# Autodesk Inventor assembly: 3_left_leg_true_final
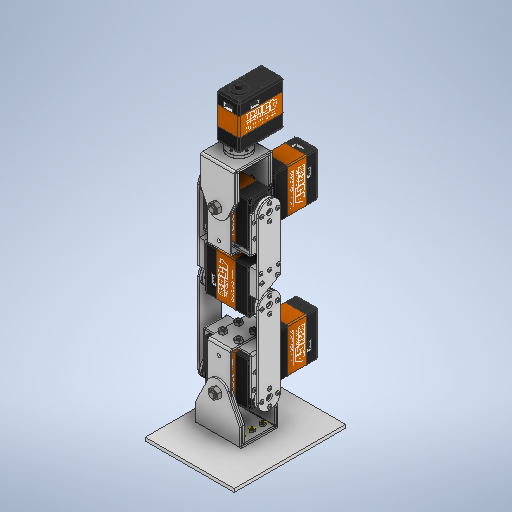
[picture p0: Inventor's stored thumbnail of the model, 512x512]
Saved by Autodesk Inventor 2026.1 (Build 301233000, 233)
## iProperties
Created: 2025-08-03
Part Number: 3_left_leg_true_final
Document SubType Name: Assembly
Designer: User
Author: User
## Documents named in this file (29)
- C:\Users\User\Documents\The Maverick's Files\College 3-3\로보인 프로젝트\RHp_Humanoid_ver1\Assembly\3_left_leg_true_final.iam
- C:\Users\User\Documents\The Maverick's Files\College 3-3\로보인 프로젝트\RHp_Humanoid_ver1\Part\HTD-45H, Horn\HTD-45H\HTD-45H.iam
- C:\Users\User\Documents\The Maverick's Files\College 3-3\로보인 프로젝트\RHp_Humanoid_ver1\Part\Frame\Leg\Left Leg\axis_1_top_frame.ipt
- C:\Users\User\Documents\The Maverick's Files\College 3-3\로보인 프로젝트\RHp_Humanoid_ver1\Part\Frame\Leg\Left Leg\axis_3_bottom_frame.ipt
- C:\Users\User\Documents\The Maverick's Files\College 3-3\로보인 프로젝트\RHp_Humanoid_ver1\Part\Frame\Leg\Left Leg\axis_2_bottom_frame.ipt
- C:\Users\User\Documents\The Maverick's Files\College 3-3\로보인 프로젝트\RHp_Humanoid_ver1\Part\Frame\Leg\Left Leg\axis_1_supplement_frame.ipt
- C:\Users\User\Documents\The Maverick's Files\College 3-3\로보인 프로젝트\RHp_Humanoid_ver1\Part\Frame\Leg\Left Leg\axis_2_4_connector_frame_powered.ipt
- C:\Users\User\Documents\The Maverick's Files\College 3-3\로보인 프로젝트\RHp_Humanoid_ver1\Part\Frame\Leg\Left Leg\axis_2_4_connector_frame_non_powered.ipt
- C:\Users\User\Documents\The Maverick's Files\College 3-3\로보인 프로젝트\RHp_Humanoid_ver1\Part\Frame\Leg\3D_printed_part_powered.ipt
- C:\Users\User\Documents\The Maverick's Files\College 3-3\로보인 프로젝트\RHp_Humanoid_ver1\Part\Frame\Leg\3D_printed_part_non_powered.ipt
- C:\Users\User\Documents\The Maverick's Files\College 3-3\로보인 프로젝트\RHp_Humanoid_ver1\Part\Frame\Leg\Left Leg\axis_4_5_connector_frame_powered.ipt
- C:\Users\User\Documents\The Maverick's Files\College 3-3\로보인 프로젝트\RHp_Humanoid_ver1\Part\Frame\Leg\Left Leg\axis_4_5_connector_frame_non_powered.ipt
- C:\Users\User\Documents\The Maverick's Files\College 3-3\로보인 프로젝트\RHp_Humanoid_ver1\Part\Frame\Leg\Left Leg\axis_5_top_frame.ipt
- C:\Users\User\Documents\The Maverick's Files\College 3-3\로보인 프로젝트\RHp_Humanoid_ver1\Part\Frame\Leg\Left Leg\axis_6_top_frame.ipt
- C:\Users\User\Documents\The Maverick's Files\College 3-3\로보인 프로젝트\RHp_Humanoid_ver1\Part\Frame\Leg\Left Leg\axis_6_bottom_frame(top).ipt
- C:\Users\User\Documents\The Maverick's Files\College 3-3\로보인 프로젝트\RHp_Humanoid_ver1\Part\Frame\Leg\Left Leg\axis_6_bottom_frame(bottom).ipt
- C:\Users\User\Documents\The Maverick's Files\College 3-3\로보인 프로젝트\RHp_Humanoid_ver1\Part\Frame\Leg\Left Leg\axis_6_supplement_frame.ipt
- C:\Users\User\Documents\The Maverick's Files\College 3-3\로보인 프로젝트\RHp_Humanoid_ver1\Part\Bolt, Bearing, Nut, Washer\볼트, 너트\볼트, 너트\M5x10 Bolt.ipt
- C:\Users\User\Documents\The Maverick's Files\College 3-3\로보인 프로젝트\RHp_Humanoid_ver1\Part\Bolt, Bearing, Nut, Washer\볼트, 너트\볼트, 너트\M5 Nylon Nut.ipt
- C:\Users\User\Documents\The Maverick's Files\College 3-3\로보인 프로젝트\RHp_Humanoid_ver1\Part\Bolt, Bearing, Nut, Washer\볼트, 너트\볼트, 너트\M3x6 Bolt.ipt
- C:\Users\User\Documents\The Maverick's Files\College 3-3\로보인 프로젝트\RHp_Humanoid_ver1\Part\Bolt, Bearing, Nut, Washer\볼트, 너트\볼트, 너트\M3 Nut.ipt
- C:\Users\User\Documents\The Maverick's Files\College 3-3\로보인 프로젝트\RHp_Humanoid_ver1\Part\Bolt, Bearing, Nut, Washer\볼트, 너트\볼트, 너트\M2x6 Bolt.ipt
- C:\Users\User\Documents\The Maverick's Files\College 3-3\로보인 프로젝트\RHp_Humanoid_ver1\Part\Bolt, Bearing, Nut, Washer\볼트, 너트\볼트, 너트\M2x4 Bolt.ipt
- C:\Users\User\Documents\The Maverick's Files\College 3-3\로보인 프로젝트\RHp_Humanoid_ver1\Part\Bolt, Bearing, Nut, Washer\볼트, 너트\볼트, 너트\M2x12 Bolt.ipt
- C:\Users\User\Documents\The Maverick's Files\College 3-3\로보인 프로젝트\RHp_Humanoid_ver1\Part\Bolt, Bearing, Nut, Washer\볼트, 너트\볼트, 너트\M2x8접시.ipt
- C:\Users\User\Documents\The Maverick's Files\College 3-3\로보인 프로젝트\RHp_Humanoid_ver1\Part\Bolt, Bearing, Nut, Washer\볼트, 너트\볼트, 너트\M2x45 Bolt.ipt
- C:\Users\User\Documents\The Maverick's Files\College 3-3\로보인 프로젝트\RHp_Humanoid_ver1\Part\HTD-45H, Horn (Silver)\HTD-45H, Horn (Silver)\Horn\Top Horn.ipt
- C:\Users\User\Documents\The Maverick's Files\College 3-3\로보인 프로젝트\RHp_Humanoid_ver1\Part\HTD-45H, Horn (Silver)\HTD-45H, Horn (Silver)\Horn\Bottom Horn.ipt
- C:\Users\User\Documents\The Maverick's Files\College 3-3\로보인 프로젝트\RHp_Humanoid_ver1\Part\Bolt, Bearing, Nut, Washer\M2 Nut.ipt
## Components (134 placed, 28 different names)
1. HTD-45H:1 [sub-assembly] — Rotational:1
2. Top Horn:1 — Rotational:1, Rigid:127
3. axis_1_top_frame:1 — Rigid:5, Rigid:29, Rigid:127, Rigid:131
4. axis_1_supplement_frame:1 — Rigid:5, Rigid:28, Rigid:83, Rigid:80, Rigid:81, Rigid:82, Rigid:84, Rigid:85, Rigid:86, Rigid:87
5. HTD-45H:3 [sub-assembly] — Rigid:25, Rotational:2
6. Top Horn:2 — Rotational:2, Rigid:128
7. Bottom Horn:2 — Rigid:130
8. axis_2_bottom_frame:1 — Rigid:25, Rigid:27, Rigid:36, Rigid:37, Rigid:38, Rigid:39, Rigid:62, Rigid:63, Rigid:64, Rigid:65, Rigid:66, Rigid:67, Rigid:68, Rigid:69, Rigid:70
9. axis_2_4_connector_frame_powered:1 — Rigid:23, Rigid:96, Rigid:97, Rigid:98, Rigid:99, Rigid:113, Rigid:114, Rigid:115, Rigid:125, Rigid:126, Rigid:128
10. axis_2_4_connector_frame_non_powered:1 — Rigid:24, Rigid:108, Rigid:109, Rigid:110, Rigid:111, Rigid:116, Rigid:117, Rigid:118, Rigid:130
11. HTD-45H:2 [sub-assembly] — Rigid:26, Rotational:3
12. Top Horn:3 — Rotational:3, Rigid:131
13. axis_3_bottom_frame:1 — Rigid:26, Rigid:27, Rigid:44, Rigid:45, Rigid:46, Rigid:47, Rigid:71, Rigid:72, Rigid:73, Rigid:74, Rigid:75
14. HTD-45H:4 [sub-assembly] — Rigid:11, Rigid:21, Rotational:4, Rotational:5
15. Top Horn:4 — Rotational:4, Rigid:132
16. Bottom Horn:4 — Rotational:5, Rigid:133
17. 3D_printed_part_powered:1 — Rigid:11, Rigid:23
18. 3D_printed_part_non_powered:1 — Rigid:21, Rigid:24
19. axis_4_5_connector_frame_powered:1 — Rigid:88, Rigid:89, Rigid:90, Rigid:91, Rigid:92, Rigid:93, Rigid:94, Rigid:95, Rigid:132, Rigid:134
20. axis_4_5_connector_frame_non_powered:1 — Rigid:100, Rigid:101, Rigid:102, Rigid:103, Rigid:104, Rigid:105, Rigid:106, Rigid:107, Rigid:133, Rigid:135
21. HTD-45H:5 [sub-assembly] — Rigid:14, Rotational:6, Rotational:7
22. Top Horn:5 — Rotational:6, Rigid:134
23. Bottom Horn:5 — Rotational:7, Rigid:135
24. axis_5_top_frame:1 — Rigid:14, Rigid:17, Rigid:48, Rigid:49, Rigid:50, Rigid:51, Rigid:52, Rigid:53, Rigid:54, Rigid:55, Rigid:56, Rigid:33, Rigid:32, Rigid:34, Rigid:35
25. HTD-45H:6 [sub-assembly] — Rigid:16, Rotational:8
26. Top Horn:6 — Rotational:8, Rigid:136
27. axis_6_top_frame:1 — Rigid:16, Rigid:17, Rigid:57, Rigid:58, Rigid:59, Rigid:60, Rigid:61, Rigid:40, Rigid:41, Rigid:42, Rigid:43
28. axis_6_supplement_frame:1 — Rigid:18, Rigid:30, Rigid:76, Rigid:77, Rigid:78, Rigid:79, Rigid:137, Rigid:138, Rigid:139, Rigid:140, Rigid:141, Rigid:142
29. axis_6_bottom_frame(top):1 — Rigid:18, Rigid:20, Rigid:31, Rigid:136
30. axis_6_bottom_frame(bottom):1 — Rigid:20, Rigid:119, Rigid:120, Rigid:121, Rigid:122, Rigid:123, Rigid:124
31. M2x4 Bolt:1 — Rigid:88
32. M2x4 Bolt:2 — Rigid:89
33. M2x4 Bolt:3 — Rigid:90
34. M2x4 Bolt:4 — Rigid:91
35. M2x4 Bolt:5 — Rigid:92
36. M2x4 Bolt:6 — Rigid:93
37. M2x4 Bolt:7 — Rigid:94
38. M2x4 Bolt:8 — Rigid:95
39. M2x4 Bolt:9 — Rigid:96
40. M2x4 Bolt:10 — Rigid:97
41. M2x4 Bolt:11 — Rigid:98
42. M2x4 Bolt:12 — Rigid:99
43. M2x4 Bolt:13 — Rigid:100
44. M2x4 Bolt:14 — Rigid:101
45. M2x4 Bolt:15 — Rigid:102
46. M2x4 Bolt:16 — Rigid:103
47. M2x4 Bolt:17 — Rigid:104
48. M2x4 Bolt:18 — Rigid:105
49. M2x4 Bolt:19 — Rigid:106
50. M2x4 Bolt:20 — Rigid:107
51. M2x4 Bolt:21 — Rigid:108
52. M2x4 Bolt:22 — Rigid:109
53. M2x4 Bolt:23 — Rigid:110
54. M2x4 Bolt:24 — Rigid:111
55. M2x6 Bolt:1 — Rigid:48
56. M2x6 Bolt:2 — Rigid:49
57. M2x6 Bolt:3 — Rigid:50
58. M2x6 Bolt:4 — Rigid:51
59. M2x6 Bolt:5 — Rigid:52
60. M2x6 Bolt:6 — Rigid:53
61. M2x6 Bolt:7 — Rigid:54
62. M2x6 Bolt:8 — Rigid:55
63. M2x6 Bolt:9 — Rigid:56
64. M2x6 Bolt:10 — Rigid:57
65. M2x6 Bolt:11 — Rigid:58
66. M2x6 Bolt:12 — Rigid:59
67. M2x6 Bolt:13 — Rigid:60
68. M2x6 Bolt:14 — Rigid:61
69. M2x6 Bolt:15 — Rigid:62
70. M2x6 Bolt:16 — Rigid:63
71. M2x6 Bolt:17 — Rigid:64
72. M2x6 Bolt:18 — Rigid:65
73. M2x6 Bolt:19 — Rigid:66
74. M2x6 Bolt:20 — Rigid:67
75. M2x6 Bolt:21 — Rigid:68
76. M2x6 Bolt:22 — Rigid:69
77. M2x6 Bolt:23 — Rigid:70
78. M2x6 Bolt:24 — Rigid:71
79. M2x6 Bolt:25 — Rigid:72
80. M2x6 Bolt:26 — Rigid:73
81. M2x6 Bolt:27 — Rigid:74
82. M2x6 Bolt:28 — Rigid:75
83. M2x6 Bolt:29 — Rigid:76
84. M2x6 Bolt:30 — Rigid:77
85. M2x6 Bolt:31 — Rigid:78
86. M2x6 Bolt:32 — Rigid:79
87. M2x6 Bolt:33 — Rigid:83
88. M2x6 Bolt:34 — Rigid:80
89. M2x6 Bolt:35 — Rigid:81
90. M2x6 Bolt:36 — Rigid:82
91. M2x6 Bolt:37 — Rigid:84
92. M2x6 Bolt:38 — Rigid:85
93. M2x6 Bolt:39 — Rigid:86
94. M2x6 Bolt:40 — Rigid:87
95. M2x8접시:1 — Rigid:119
96. M2x8접시:2 — Rigid:120
97. M2x8접시:3 — Rigid:121
98. M2x8접시:4 — Rigid:122
99. M2x8접시:5 — Rigid:123
100. M2x8접시:6 — Rigid:124
101. M2x12 Bolt:1 — Rigid:113
102. M2x12 Bolt:2 — Rigid:114
103. M2x12 Bolt:3 — Rigid:115
104. M2x12 Bolt:4 — Rigid:116
105. M2x12 Bolt:5 — Rigid:117
106. M2x12 Bolt:6 — Rigid:118
107. M2x45 Bolt:1 — Rigid:125
108. M2x45 Bolt:2 — Rigid:126
109. M2 Nut:1 — Rigid:137
110. M2 Nut:2 — Rigid:138
111. M2 Nut:3 — Rigid:139
112. M2 Nut:4 — Rigid:140
113. M2 Nut:5 — Rigid:141
114. M2 Nut:6 — Rigid:142
115. M3x6 Bolt:1 — Rigid:33
116. M3x6 Bolt:2 — Rigid:32
117. M3x6 Bolt:3 — Rigid:34
118. M3x6 Bolt:4 — Rigid:35
119. M3x6 Bolt:5 — Rigid:36
120. M3x6 Bolt:6 — Rigid:37
121. M3x6 Bolt:7 — Rigid:38
122. M3x6 Bolt:8 — Rigid:39
123. M3 Nut:1 — Rigid:40
124. M3 Nut:2 — Rigid:41
125. M3 Nut:3 — Rigid:42
126. M3 Nut:4 — Rigid:43
127. M3 Nut:5 — Rigid:44
128. M3 Nut:6 — Rigid:45
129. M3 Nut:7 — Rigid:46
130. M3 Nut:8 — Rigid:47
131. M5x10 Bolt:1 — Rigid:30
132. M5x10 Bolt:4 — Rigid:28
133. M5 Nylon Nut:1 — Rigid:29
134. M5 Nylon Nut:2 — Rigid:31
## Relationships (134: WeldJoint 126, RevoluteJoint 8)
- Rigid:5 [WeldJoint]: axis_1_top_frame:1 ↔ axis_1_supplement_frame:1
- Rigid:11 [WeldJoint]: HTD-45H:4 ↔ 3D_printed_part_powered:1
- Rigid:14 [WeldJoint]: HTD-45H:5 ↔ axis_5_top_frame:1
- Rigid:16 [WeldJoint]: HTD-45H:6 ↔ axis_6_top_frame:1
- Rigid:17 [WeldJoint]: axis_5_top_frame:1 ↔ axis_6_top_frame:1
- Rigid:18 [WeldJoint]: axis_6_supplement_frame:1 ↔ axis_6_bottom_frame(top):1
- Rigid:20 [WeldJoint]: axis_6_bottom_frame(top):1 ↔ axis_6_bottom_frame(bottom):1
- Rigid:21 [WeldJoint]: HTD-45H:4 ↔ 3D_printed_part_non_powered:1
- Rigid:23 [WeldJoint]: axis_2_4_connector_frame_powered:1 ↔ 3D_printed_part_powered:1
- Rigid:24 [WeldJoint]: axis_2_4_connector_frame_non_powered:1 ↔ 3D_printed_part_non_powered:1
- Rigid:25 [WeldJoint]: HTD-45H:3 ↔ axis_2_bottom_frame:1
- Rigid:26 [WeldJoint]: HTD-45H:2 ↔ axis_3_bottom_frame:1
- Rigid:27 [WeldJoint]: axis_2_bottom_frame:1 ↔ axis_3_bottom_frame:1
- Rigid:28 [WeldJoint]: axis_1_supplement_frame:1 ↔ M5x10 Bolt:4
- Rigid:29 [WeldJoint]: axis_1_top_frame:1 ↔ M5 Nylon Nut:1
- Rigid:30 [WeldJoint]: axis_6_supplement_frame:1 ↔ M5x10 Bolt:1
- Rigid:31 [WeldJoint]: axis_6_bottom_frame(top):1 ↔ M5 Nylon Nut:2
- Rigid:32 [WeldJoint]: axis_5_top_frame:1 ↔ M3x6 Bolt:2
- Rigid:33 [WeldJoint]: axis_5_top_frame:1 ↔ M3x6 Bolt:1
- Rigid:34 [WeldJoint]: axis_5_top_frame:1 ↔ M3x6 Bolt:3
- Rigid:35 [WeldJoint]: axis_5_top_frame:1 ↔ M3x6 Bolt:4
- Rigid:36 [WeldJoint]: axis_2_bottom_frame:1 ↔ M3x6 Bolt:5
- Rigid:37 [WeldJoint]: axis_2_bottom_frame:1 ↔ M3x6 Bolt:6
- Rigid:38 [WeldJoint]: axis_2_bottom_frame:1 ↔ M3x6 Bolt:7
- Rigid:39 [WeldJoint]: axis_2_bottom_frame:1 ↔ M3x6 Bolt:8
- Rigid:40 [WeldJoint]: axis_6_top_frame:1 ↔ M3 Nut:1
- Rigid:41 [WeldJoint]: axis_6_top_frame:1 ↔ M3 Nut:2
- Rigid:42 [WeldJoint]: axis_6_top_frame:1 ↔ M3 Nut:3
- Rigid:43 [WeldJoint]: axis_6_top_frame:1 ↔ M3 Nut:4
- Rigid:44 [WeldJoint]: axis_3_bottom_frame:1 ↔ M3 Nut:5
- Rigid:45 [WeldJoint]: axis_3_bottom_frame:1 ↔ M3 Nut:6
- Rigid:46 [WeldJoint]: axis_3_bottom_frame:1 ↔ M3 Nut:7
- Rigid:47 [WeldJoint]: axis_3_bottom_frame:1 ↔ M3 Nut:8
- Rigid:48 [WeldJoint]: axis_5_top_frame:1 ↔ M2x6 Bolt:1
- Rigid:49 [WeldJoint]: axis_5_top_frame:1 ↔ M2x6 Bolt:2
- Rigid:50 [WeldJoint]: axis_5_top_frame:1 ↔ M2x6 Bolt:3
- Rigid:51 [WeldJoint]: axis_5_top_frame:1 ↔ M2x6 Bolt:4
- Rigid:52 [WeldJoint]: axis_5_top_frame:1 ↔ M2x6 Bolt:5
- Rigid:53 [WeldJoint]: axis_5_top_frame:1 ↔ M2x6 Bolt:6
- Rigid:54 [WeldJoint]: axis_5_top_frame:1 ↔ M2x6 Bolt:7
- Rigid:55 [WeldJoint]: axis_5_top_frame:1 ↔ M2x6 Bolt:8
- Rigid:56 [WeldJoint]: axis_5_top_frame:1 ↔ M2x6 Bolt:9
- Rigid:57 [WeldJoint]: axis_6_top_frame:1 ↔ M2x6 Bolt:10
- Rigid:58 [WeldJoint]: axis_6_top_frame:1 ↔ M2x6 Bolt:11
- Rigid:59 [WeldJoint]: axis_6_top_frame:1 ↔ M2x6 Bolt:12
- Rigid:60 [WeldJoint]: axis_6_top_frame:1 ↔ M2x6 Bolt:13
- Rigid:61 [WeldJoint]: axis_6_top_frame:1 ↔ M2x6 Bolt:14
- Rigid:62 [WeldJoint]: axis_2_bottom_frame:1 ↔ M2x6 Bolt:15
- Rigid:63 [WeldJoint]: axis_2_bottom_frame:1 ↔ M2x6 Bolt:16
- Rigid:64 [WeldJoint]: axis_2_bottom_frame:1 ↔ M2x6 Bolt:17
- Rigid:65 [WeldJoint]: axis_2_bottom_frame:1 ↔ M2x6 Bolt:18
- Rigid:66 [WeldJoint]: axis_2_bottom_frame:1 ↔ M2x6 Bolt:19
- Rigid:67 [WeldJoint]: axis_2_bottom_frame:1 ↔ M2x6 Bolt:20
- Rigid:68 [WeldJoint]: axis_2_bottom_frame:1 ↔ M2x6 Bolt:21
- Rigid:69 [WeldJoint]: axis_2_bottom_frame:1 ↔ M2x6 Bolt:22
- Rigid:70 [WeldJoint]: axis_2_bottom_frame:1 ↔ M2x6 Bolt:23
- Rigid:71 [WeldJoint]: axis_3_bottom_frame:1 ↔ M2x6 Bolt:24
- Rigid:72 [WeldJoint]: axis_3_bottom_frame:1 ↔ M2x6 Bolt:25
- Rigid:73 [WeldJoint]: axis_3_bottom_frame:1 ↔ M2x6 Bolt:26
- Rigid:74 [WeldJoint]: axis_3_bottom_frame:1 ↔ M2x6 Bolt:27
- Rigid:75 [WeldJoint]: axis_3_bottom_frame:1 ↔ M2x6 Bolt:28
- Rigid:76 [WeldJoint]: axis_6_supplement_frame:1 ↔ M2x6 Bolt:29
- Rigid:77 [WeldJoint]: axis_6_supplement_frame:1 ↔ M2x6 Bolt:30
- Rigid:78 [WeldJoint]: axis_6_supplement_frame:1 ↔ M2x6 Bolt:31
- Rigid:79 [WeldJoint]: axis_6_supplement_frame:1 ↔ M2x6 Bolt:32
- Rigid:83 [WeldJoint]: axis_1_supplement_frame:1 ↔ M2x6 Bolt:33
- Rigid:80 [WeldJoint]: axis_1_supplement_frame:1 ↔ M2x6 Bolt:34
- Rigid:81 [WeldJoint]: axis_1_supplement_frame:1 ↔ M2x6 Bolt:35
- Rigid:82 [WeldJoint]: axis_1_supplement_frame:1 ↔ M2x6 Bolt:36
- Rigid:84 [WeldJoint]: axis_1_supplement_frame:1 ↔ M2x6 Bolt:37
- Rigid:85 [WeldJoint]: axis_1_supplement_frame:1 ↔ M2x6 Bolt:38
- Rigid:86 [WeldJoint]: axis_1_supplement_frame:1 ↔ M2x6 Bolt:39
- Rigid:87 [WeldJoint]: axis_1_supplement_frame:1 ↔ M2x6 Bolt:40
- Rigid:88 [WeldJoint]: axis_4_5_connector_frame_powered:1 ↔ M2x4 Bolt:1
- Rigid:89 [WeldJoint]: axis_4_5_connector_frame_powered:1 ↔ M2x4 Bolt:2
- Rigid:90 [WeldJoint]: axis_4_5_connector_frame_powered:1 ↔ M2x4 Bolt:3
- Rigid:91 [WeldJoint]: axis_4_5_connector_frame_powered:1 ↔ M2x4 Bolt:4
- Rigid:92 [WeldJoint]: axis_4_5_connector_frame_powered:1 ↔ M2x4 Bolt:5
- Rigid:93 [WeldJoint]: axis_4_5_connector_frame_powered:1 ↔ M2x4 Bolt:6
- Rigid:94 [WeldJoint]: axis_4_5_connector_frame_powered:1 ↔ M2x4 Bolt:7
- Rigid:95 [WeldJoint]: axis_4_5_connector_frame_powered:1 ↔ M2x4 Bolt:8
- Rigid:96 [WeldJoint]: axis_2_4_connector_frame_powered:1 ↔ M2x4 Bolt:9
- Rigid:97 [WeldJoint]: axis_2_4_connector_frame_powered:1 ↔ M2x4 Bolt:10
- Rigid:98 [WeldJoint]: axis_2_4_connector_frame_powered:1 ↔ M2x4 Bolt:11
- Rigid:99 [WeldJoint]: axis_2_4_connector_frame_powered:1 ↔ M2x4 Bolt:12
- Rigid:100 [WeldJoint]: axis_4_5_connector_frame_non_powered:1 ↔ M2x4 Bolt:13
- Rigid:101 [WeldJoint]: axis_4_5_connector_frame_non_powered:1 ↔ M2x4 Bolt:14
- Rigid:102 [WeldJoint]: axis_4_5_connector_frame_non_powered:1 ↔ M2x4 Bolt:15
- Rigid:103 [WeldJoint]: axis_4_5_connector_frame_non_powered:1 ↔ M2x4 Bolt:16
- Rigid:104 [WeldJoint]: axis_4_5_connector_frame_non_powered:1 ↔ M2x4 Bolt:17
- Rigid:105 [WeldJoint]: axis_4_5_connector_frame_non_powered:1 ↔ M2x4 Bolt:18
- Rigid:106 [WeldJoint]: axis_4_5_connector_frame_non_powered:1 ↔ M2x4 Bolt:19
- Rigid:107 [WeldJoint]: axis_4_5_connector_frame_non_powered:1 ↔ M2x4 Bolt:20
- Rigid:108 [WeldJoint]: axis_2_4_connector_frame_non_powered:1 ↔ M2x4 Bolt:21
- Rigid:109 [WeldJoint]: axis_2_4_connector_frame_non_powered:1 ↔ M2x4 Bolt:22
- Rigid:110 [WeldJoint]: axis_2_4_connector_frame_non_powered:1 ↔ M2x4 Bolt:23
- Rigid:111 [WeldJoint]: axis_2_4_connector_frame_non_powered:1 ↔ M2x4 Bolt:24
- Rigid:113 [WeldJoint]: axis_2_4_connector_frame_powered:1 ↔ M2x12 Bolt:1
- Rigid:114 [WeldJoint]: axis_2_4_connector_frame_powered:1 ↔ M2x12 Bolt:2
- Rigid:115 [WeldJoint]: axis_2_4_connector_frame_powered:1 ↔ M2x12 Bolt:3
- Rigid:116 [WeldJoint]: axis_2_4_connector_frame_non_powered:1 ↔ M2x12 Bolt:4
- Rigid:117 [WeldJoint]: axis_2_4_connector_frame_non_powered:1 ↔ M2x12 Bolt:5
- Rigid:118 [WeldJoint]: axis_2_4_connector_frame_non_powered:1 ↔ M2x12 Bolt:6
- Rigid:119 [WeldJoint]: axis_6_bottom_frame(bottom):1 ↔ M2x8접시:1
- Rigid:120 [WeldJoint]: axis_6_bottom_frame(bottom):1 ↔ M2x8접시:2
- Rigid:121 [WeldJoint]: axis_6_bottom_frame(bottom):1 ↔ M2x8접시:3
- Rigid:122 [WeldJoint]: axis_6_bottom_frame(bottom):1 ↔ M2x8접시:4
- Rigid:123 [WeldJoint]: axis_6_bottom_frame(bottom):1 ↔ M2x8접시:5
- Rigid:124 [WeldJoint]: axis_6_bottom_frame(bottom):1 ↔ M2x8접시:6
- Rigid:125 [WeldJoint]: axis_2_4_connector_frame_powered:1 ↔ M2x45 Bolt:1
- Rigid:126 [WeldJoint]: axis_2_4_connector_frame_powered:1 ↔ M2x45 Bolt:2
- Rotational:1 [RevoluteJoint]: HTD-45H:1 ↔ Top Horn:1
- Rigid:127 [WeldJoint]: Top Horn:1 ↔ axis_1_top_frame:1
- Rotational:2 [RevoluteJoint]: HTD-45H:3 ↔ Top Horn:2
- Rigid:128 [WeldJoint]: Top Horn:2 ↔ axis_2_4_connector_frame_powered:1
- Rigid:130 [WeldJoint]: Bottom Horn:2 ↔ axis_2_4_connector_frame_non_powered:1
- Rotational:3 [RevoluteJoint]: HTD-45H:2 ↔ Top Horn:3
- Rigid:131 [WeldJoint]: axis_1_top_frame:1 ↔ Top Horn:3
- Rotational:4 [RevoluteJoint]: HTD-45H:4 ↔ Top Horn:4
- Rotational:5 [RevoluteJoint]: HTD-45H:4 ↔ Bottom Horn:4
- Rigid:132 [WeldJoint]: Top Horn:4 ↔ axis_4_5_connector_frame_powered:1
- Rigid:133 [WeldJoint]: Bottom Horn:4 ↔ axis_4_5_connector_frame_non_powered:1
- Rotational:6 [RevoluteJoint]: HTD-45H:5 ↔ Top Horn:5
- Rotational:7 [RevoluteJoint]: HTD-45H:5 ↔ Bottom Horn:5
- Rigid:134 [WeldJoint]: axis_4_5_connector_frame_powered:1 ↔ Top Horn:5
- Rigid:135 [WeldJoint]: axis_4_5_connector_frame_non_powered:1 ↔ Bottom Horn:5
- Rotational:8 [RevoluteJoint]: HTD-45H:6 ↔ Top Horn:6
- Rigid:136 [WeldJoint]: Top Horn:6 ↔ axis_6_bottom_frame(top):1
- Rigid:137 [WeldJoint]: axis_6_supplement_frame:1 ↔ M2 Nut:1
- Rigid:138 [WeldJoint]: axis_6_supplement_frame:1 ↔ M2 Nut:2
- Rigid:139 [WeldJoint]: axis_6_supplement_frame:1 ↔ M2 Nut:3
- Rigid:140 [WeldJoint]: axis_6_supplement_frame:1 ↔ M2 Nut:4
- Rigid:141 [WeldJoint]: axis_6_supplement_frame:1 ↔ M2 Nut:5
- Rigid:142 [WeldJoint]: axis_6_supplement_frame:1 ↔ M2 Nut:6
